# Autodesk Inventor assembly: Foot
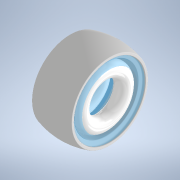
[picture p0: Inventor's stored thumbnail of the model, 180x180]
Saved by Autodesk Inventor 2022.2 (Build 262287000, 287)
## iProperties
Created: 2021-12-28
Part Number: Foot
Document SubType Name: Assembly
Designer: Jochen
Author: Jochen
## Documents named in this file (4)
- D:\Projects\Chewbacca\CAD\foot\Foot.iam
- D:\Projects\Chewbacca\CAD\foot\Toe.ipt
- D:\Projects\Chewbacca\CAD\foot\ToeSilikoneRubber.ipt
- D:\Projects\Chewbacca\CAD\foot\ToePalm.ipt
## Components (4 placed, 3 different names)
1. Toe:1 — Mate:7, Mate:8, Mate:9, Mate:10, Mate:11, Mate:12, Mate:14, Mate:15
2. ToeSilikoneRubber:1 — Mate:10, Mate:11, Mate:13, Mate:14
3. ToeSilikoneRubber:2 — Mate:12, Mate:13, Mate:15
4. ToePalm:1 — Mate:7, Mate:8, Mate:9
## Relationships (9: Mate 9)
- Mate:7: Toe:1 ↔ ToePalm:1
- Mate:8: Toe:1 ↔ ToePalm:1
- Mate:9: Toe:1 ↔ ToePalm:1
- Mate:10: Toe:1 ↔ ToeSilikoneRubber:1
- Mate:11: Toe:1 ↔ ToeSilikoneRubber:1
- Mate:12: Toe:1 ↔ ToeSilikoneRubber:2
- Mate:13: ToeSilikoneRubber:1 ↔ ToeSilikoneRubber:2
- Mate:14 (-4.75 mm): Toe:1 ↔ ToeSilikoneRubber:1
- Mate:15 (-4.75 mm): Toe:1 ↔ ToeSilikoneRubber:2
